# Autodesk Inventor assembly: Base assembly
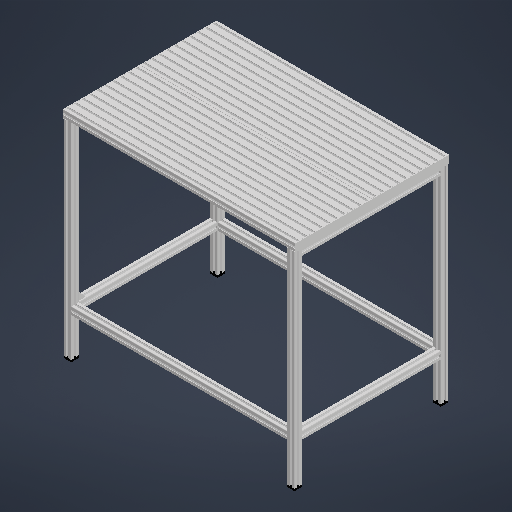
[picture p0: Inventor's stored thumbnail of the model, 512x512]
Saved by Autodesk Inventor 2027 (Build 310192000, 192)
## iProperties
Created: 2026-04-15
Part Number: Base assembly
Document SubType Name: Assembly
Designer: ratik
Author: ratik
## Documents named in this file (8)
- C:\Users\ratik\OneDrive\Personal Folder\00_Startup\01_Mectosys_Prototype\01_Prototype\01_Mechanical\3D file\Assembly File\Base assembly.iam
- C:\Users\ratik\OneDrive\Personal Folder\00_Startup\01_Mectosys_Prototype\01_Prototype\01_Mechanical\3D file\01_Station Table\01_EFSP6-30030-900_Inventor\EFSP6-30030-900.ipt
- C:\Users\ratik\OneDrive\Personal Folder\00_Startup\01_Mectosys_Prototype\01_Prototype\01_Mechanical\3D file\01_Station Table\02_HFS6-3030-2400_Inventor\HFS6-3030-800.ipt
- C:\Users\ratik\OneDrive\Personal Folder\00_Startup\01_Mectosys_Prototype\01_Prototype\01_Mechanical\3D file\01_Station Table\02_HFS6-3030-2400_Inventor\HFS6-3030-540.ipt
- C:\Users\ratik\OneDrive\Personal Folder\00_Startup\01_Mectosys_Prototype\01_Prototype\01_Mechanical\3D file\01_Station Table\02_HFS6-3030-2400_Inventor\HFS6-3030-840.ipt
- C:\Users\ratik\OneDrive\Personal Folder\00_Startup\01_Mectosys_Prototype\01_Prototype\01_Mechanical\3D file\01_Station Table\03_CHBLFSN6_Inventor\BRACKET_CHBLFSN6.ipt
- C:\Users\ratik\OneDrive\Personal Folder\00_Startup\01_Mectosys_Prototype\01_Prototype\01_Mechanical\3D file\01_Station Table\06_HFPD6-3030_STEP_AP214_20260415\HFPD6-3030\HFPD6-3030.ipt
- C:\Users\ratik\OneDrive\Personal Folder\00_Startup\01_Mectosys_Prototype\01_Prototype\01_Mechanical\3D file\01_Station Table\07_HFC6-3090-B_Inventor\HFC6-3090-B.ipt
## Components (31 placed, 7 different names)
1. EFSP6-30030-900:1 — Mate:1, Flush:1, Flush:2, Mate:3, Flush:5, Flush:6, Mate:4, Mate:6, Flush:7, Mate:14, Flush:13, Mate:15
2. EFSP6-30030-900:2 — Mate:1, Flush:1, Flush:2, Mate:2, Flush:3, Flush:4, Mate:16, Flush:14, Mate:17
3. BRACKET_CHBLFSN6:1 — Mate:10, Mate:11, Mate:12
4. HFS6-3030-800:1 — Mate:2, Flush:3, Flush:4, Mate:8, Flush:10, Mate:9
5. HFS6-3030-800:2 — Flush:8, Flush:11, Flush:12, Mate:13
6. HFS6-3030-800:3 — Mate:3, Flush:5, Flush:6, Mate:4, Mate:7
7. HFS6-3030-800:4 — Mate:5, Flush:9, Mate:11
8. HFS6-3030-540:1 — Mate:5, Mate:6, Flush:7
9. HFS6-3030-540:2
10. HFS6-3030-540:3 — Mate:7, Flush:8, Flush:9, Mate:10, Mate:12
11. HFS6-3030-540:4
12. HFS6-3030-840:1 — Mate:8, Flush:10, Mate:9
13. HFS6-3030-840:2
14. HFPD6-3030:1 — Flush:11, Flush:12, Mate:13
15. HFPD6-3030:2
16. HFPD6-3030:3
17. HFPD6-3030:4
18. HFC6-3090-B:1 — Mate:14, Flush:13, Mate:15
19. HFC6-3090-B:2
20. HFC6-3090-B:3
21. HFC6-3090-B:4
22. HFC6-3090-B:5
23. HFC6-3090-B:6
24. HFC6-3090-B:7
25. HFC6-3090-B:8 — Mate:16, Flush:14, Mate:17
26. HFC6-3090-B:9
27. HFC6-3090-B:10
28. HFC6-3090-B:11
29. HFC6-3090-B:12
30. HFC6-3090-B:13
31. HFC6-3090-B:14
## Component patterns: (2 elements, first: HFS6-3030-800:1), (2 elements, first: HFS6-3030-800:3), (2 elements, first: HFS6-3030-540:1), (2 elements, first: HFS6-3030-540:3), (2 elements, first: HFS6-3030-840:1), (4 elements, first: HFPD6-3030:1), (7 elements, first: HFC6-3090-B:1), (7 elements, first: HFC6-3090-B:8)
## Relationships (31: Mate 17, Flush 14)
- Mate:1: EFSP6-30030-900:1 ↔ EFSP6-30030-900:2
- Flush:1: EFSP6-30030-900:1 ↔ EFSP6-30030-900:2
- Flush:2: EFSP6-30030-900:1 ↔ EFSP6-30030-900:2
- Mate:2: EFSP6-30030-900:2 ↔ HFS6-3030-800:1
- Flush:3: EFSP6-30030-900:2 ↔ HFS6-3030-800:1
- Flush:4: EFSP6-30030-900:2 ↔ HFS6-3030-800:1
- Mate:3: EFSP6-30030-900:1 ↔ HFS6-3030-800:3
- Flush:5: EFSP6-30030-900:1 ↔ HFS6-3030-800:3
- Flush:6: EFSP6-30030-900:1 ↔ HFS6-3030-800:3
- Mate:4: EFSP6-30030-900:1 ↔ HFS6-3030-800:3
- Mate:5: HFS6-3030-800:4 ↔ HFS6-3030-540:1
- Mate:6: EFSP6-30030-900:1 ↔ HFS6-3030-540:1
- Flush:7: EFSP6-30030-900:1 ↔ HFS6-3030-540:1
- Mate:7: HFS6-3030-800:3 ↔ HFS6-3030-540:3
- Flush:8 (150 mm): HFS6-3030-800:2 ↔ HFS6-3030-540:3
- Flush:9: HFS6-3030-800:4 ↔ HFS6-3030-540:3
- Mate:8: HFS6-3030-800:1 ↔ HFS6-3030-840:1
- Flush:10: HFS6-3030-800:1 ↔ HFS6-3030-840:1
- Mate:9 (150 mm): HFS6-3030-800:1 ↔ HFS6-3030-840:1
- Mate:10: BRACKET_CHBLFSN6:1 ↔ HFS6-3030-540:3
- Mate:11: BRACKET_CHBLFSN6:1 ↔ HFS6-3030-800:4
- Mate:12 (5 mm): BRACKET_CHBLFSN6:1 ↔ HFS6-3030-540:3
- Flush:11: HFS6-3030-800:2 ↔ HFPD6-3030:1
- Flush:12: HFS6-3030-800:2 ↔ HFPD6-3030:1
- Mate:13: HFS6-3030-800:2 ↔ HFPD6-3030:1
- Mate:14: EFSP6-30030-900:1 ↔ HFC6-3090-B:1
- Flush:13: EFSP6-30030-900:1 ↔ HFC6-3090-B:1
- Mate:15: EFSP6-30030-900:1 ↔ HFC6-3090-B:1
- Mate:16: EFSP6-30030-900:2 ↔ HFC6-3090-B:8
- Flush:14: EFSP6-30030-900:2 ↔ HFC6-3090-B:8
- Mate:17: EFSP6-30030-900:2 ↔ HFC6-3090-B:8
